# Autodesk Inventor assembly: Ensamblaje carcasa superior
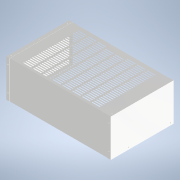
[picture p0: Inventor's stored thumbnail of the model, 180x180]
Saved by Autodesk Inventor 2021 (Build 250183000, 183)
## iProperties
Created: 2021-04-15
Part Number: Ensamblaje carcasa superior
Document SubType Name: Assembly
Designer: Admin
Mass: 3427.14 g
Surface Area: 11666.5 cm^2
Volume: 435.358 cm^3
Density: 7.872 g/cm^3
Author: Admin
## Documents named in this file (10)
- D:\Nelson\Documentos\Inventor\Proyecto_PAI\Ensamblaje carcasa superior.iam
- D:\Nelson\Documentos\Inventor\Proyecto_PAI\Tapa_superior_superior.ipt
- D:\Nelson\Documentos\Inventor\Proyecto_PAI\Tapa_superior_izquierda.ipt
- D:\Nelson\Documentos\Inventor\Proyecto_PAI\Tapa_superior_derecha.ipt
- D:\Nelson\Documentos\Inventor\Proyecto_PAI\Ensamblaje carcasa superior\AIP\FEA\dlmx15q80.fins
- D:\Nelson\Documentos\Inventor\Proyecto_PAI\Ensamblaje carcasa superior\AIP\FEA\dlmx15qrk.fsat
- D:\Nelson\Documentos\Inventor\Proyecto_PAI\Ensamblaje carcasa superior\AIP\FEA\dlmx15qrk.ftes
- D:\Nelson\Documentos\Inventor\Proyecto_PAI\Ensamblaje carcasa superior\AIP\FEA\dlmx15qsg.fwiz
- D:\Nelson\Documentos\Inventor\Proyecto_PAI\Ensamblaje carcasa superior\AIP\FEA\dlmx15r0g.fmsh
- D:\Nelson\Documentos\Inventor\Proyecto_PAI\Ensamblaje carcasa superior\AIP\FEA\dlmx15r0h.fres
## Components (3 placed, 3 different names)
1. Tapa_superior_superior:1 — Coincidencia:1, Coincidencia:2, Coincidencia:3, Coincidencia:4, Coincidencia:5, Coincidencia:6
2. Tapa_superior_izquierda:1 — Coincidencia:1, Coincidencia:2, Coincidencia:3
3. Tapa_superior_derecha:1 — Coincidencia:4, Coincidencia:5, Coincidencia:6
## Relationships (6: Mate 6)
- Coincidencia:1 [Mate]: Tapa_superior_superior:1 ↔ Tapa_superior_izquierda:1
- Coincidencia:2 [Mate]: Tapa_superior_superior:1 ↔ Tapa_superior_izquierda:1
- Coincidencia:3 [Mate]: Tapa_superior_superior:1 ↔ Tapa_superior_izquierda:1
- Coincidencia:4 [Mate]: Tapa_superior_superior:1 ↔ Tapa_superior_derecha:1
- Coincidencia:5 [Mate]: Tapa_superior_superior:1 ↔ Tapa_superior_derecha:1
- Coincidencia:6 [Mate]: Tapa_superior_superior:1 ↔ Tapa_superior_derecha:1
## Named parameters: sa_0 = 0, sa_1 = 0, sa_2 = -981
note: some values were not read from the file. Shown as the stored number, unit unknown: "sa_0", "sa_1", "sa_2".
